# Autodesk Inventor assembly: shoot
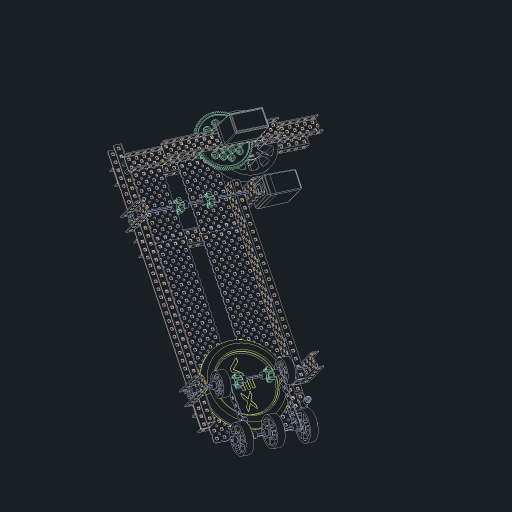
[picture p0: Inventor's stored thumbnail of the model, 512x512]
Saved by Autodesk Inventor 2023 (Build 270158000, 158)
## iProperties
Created: 2023-03-08
Part Number: shoot
Document SubType Name: Assembly
Designer: Windows Macbook
Author: Windows Macbook
## Documents named in this file (39)
- C:\Users\Windows Macbook\Desktop\VRC-SPIN-UP\Inventor\Assembly\Pre Worlds\V1\shoot.iam
- C:\Users\Windows Macbook\Desktop\VRC-SPIN-UP\Inventor\Structure\C Channel\Aluminum 1x2x1\Alu C 1x2x1x35.ipt
- C:\Users\Windows Macbook\Desktop\VRC-SPIN-UP\Inventor\Structure\C Channel\Aluminum 1x2x1\Alu C 1x2x1x14.ipt
- C:\Users\Windows Macbook\Desktop\VRC-SPIN-UP\Inventor\Structure\Plate\Steel\Steel Plate 5x25.ipt
- C:\Users\Windows Macbook\Desktop\VRC-SPIN-UP\Inventor\Structure\Plate\Steel\Steel Plate 5x10.ipt
- C:\Users\Windows Macbook\Desktop\VRC-SPIN-UP\Inventor\Structure\C Channel\Aluminum 1x2x1\Alu C 1x2x1x25.ipt
- C:\Users\Windows Macbook\Desktop\VRC-SPIN-UP\Inventor\Motion\Wheels\Flex Wheels\4 Flex, LS.iam
- C:\Users\Windows Macbook\Desktop\VRC-SPIN-UP\Inventor\Structure\Standoff\Standoff .50.ipt
- C:\Users\Windows Macbook\Desktop\VRC-SPIN-UP\Inventor\Structure\Standoff.ipt
- C:\Users\Windows Macbook\Desktop\VRC-SPIN-UP\Inventor\Structure\C Channel\Aluminum 1x3x1\Alu C 1x3x1x14.ipt
- C:\Users\Windows Macbook\Desktop\VRC-SPIN-UP\Inventor\Motion\Spacers\Spacer Nylon .375 OD\NSpacer .375 OD x .500.ipt
- C:\Users\Windows Macbook\Desktop\VRC-SPIN-UP\Inventor\Motion\Spacers\Spacer Nylon .375 OD.ipt
- C:\Users\Windows Macbook\Desktop\VRC-SPIN-UP\Inventor\Motion\Spacers\Spacer Nylon .375 OD\NSpacer .375 OD x .250.ipt
- C:\Users\Windows Macbook\Desktop\VRC-SPIN-UP\Inventor\Structure\Hardware\Screw Steel - Star.ipt
- C:\Users\Windows Macbook\Desktop\VRC-SPIN-UP\Inventor\Structure\Hardware\Screw Steel - Star\SScrew Star Smooth 1.000.ipt
- C:\Users\Windows Macbook\Desktop\VRC-SPIN-UP\Inventor\Structure\Hardware\Nut Nylock.ipt
- C:\Users\Windows Macbook\Desktop\VRC-SPIN-UP\Inventor\Motion\Shaft LS\Bearing Flat.ipt
- C:\Users\Windows Macbook\Desktop\VRC-SPIN-UP\Inventor\Motion\Spacers\Spacer Nylon .313 OD.ipt
- C:\Users\Windows Macbook\Desktop\VRC-SPIN-UP\Inventor\Motion\Gears\HS Gear\HS 12T Gear, Square.iam
- C:\Users\Windows Macbook\Desktop\VRC-SPIN-UP\Inventor\Motion\Gears\HS Gear.iam
- C:\Users\Windows Macbook\Desktop\VRC-SPIN-UP\Inventor\Motion\Gears\LS 84T Gear.ipt
- C:\Users\Windows Macbook\Desktop\VRC-SPIN-UP\Inventor\Motion\Spacers\Spacer Nylon .313 OD\NSpacer .313 OD x .125.ipt
- C:\Users\Windows Macbook\Desktop\VRC-SPIN-UP\Inventor\Motion\Spacers\Spacer Nylon .313 OD\NSpacer .313 OD x .250.ipt
- C:\Users\Windows Macbook\Desktop\VRC-SPIN-UP\Inventor\Structure\Standoff\Standoff 1.00.ipt
- C:\Users\Windows Macbook\Desktop\VRC-SPIN-UP\Inventor\Structure\C Channel\Aluminum 1x2x1\Alu C 1x2x1x15.ipt
- C:\Users\Windows Macbook\Desktop\VRC-SPIN-UP\Inventor\Structure\Plate\Steel\Steel Plate 1x8.ipt
- C:\Users\Windows Macbook\Desktop\VRC-SPIN-UP\Inventor\Disk.ipt
- C:\Users\Windows Macbook\Desktop\VRC-SPIN-UP\Inventor\Structure\C Channel\Aluminum 1x2x1\Alu C 1x2x1x5.ipt
- C:\Users\Windows Macbook\Desktop\VRC-SPIN-UP\Inventor\Motion\Shaft LS\Shaft LS\Shaft LS 8.0.ipt
- C:\Users\Windows Macbook\Desktop\VRC-SPIN-UP\Inventor\Motion\Shaft LS\Shaft LS.ipt
- C:\Users\Windows Macbook\Desktop\VRC-SPIN-UP\Inventor\Motion\Wheels\Flex Wheels\1.625 Flex, LS.iam
- C:\Users\Windows Macbook\Desktop\VRC-SPIN-UP\Inventor\Motion\Reference Files\Shaft Collar Metal.ipt
- C:\Users\Windows Macbook\Desktop\VRC-SPIN-UP\Inventor\Motion\Wheels\Flex Wheels\2 Flex, LS.iam
- C:\Users\Windows Macbook\Desktop\VRC-SPIN-UP\Inventor\Motion\Shaft LS\Shaft LS\Shaft LS 5.5.ipt
- C:\Users\Windows Macbook\Desktop\VRC-SPIN-UP\Inventor\Motion\Sprockets\9P Sprocket.iam
- C:\Users\Windows Macbook\Desktop\VRC-SPIN-UP\Inventor\Motion\Spacers\Spacer Nylon .313 OD\NSpacer .313 OD x .375.ipt
- C:\Users\Windows Macbook\Desktop\VRC-SPIN-UP\Inventor\Motion\Sprockets\9P Sprocket\9P 6T Sprocket, Square.iam
- C:\Users\Windows Macbook\Desktop\VRC-SPIN-UP\Inventor\Electronics\V5 Simple Motor.ipt
- C:\Users\Windows Macbook\Desktop\VRC-SPIN-UP\Inventor\Structure\Standoff\Standoff .75.ipt
## Components (94 placed, 31 different names)
1. Alu C 1x2x1x35:1 — Insert:1, Insert:2, Insert:15, Insert:16, Insert:18, Insert:19, Insert:22, Insert:23, Insert:43, Insert:44, Insert:91, Insert:92
2. Alu C 1x2x1x25:1 — Insert:17, Insert:113, Insert:117, Insert:118
3. Alu C 1x2x1x14:2 — Insert:1, Insert:2, Insert:7, Insert:8, Insert:9, Insert:10, Insert:24, Insert:26
4. Alu C 1x2x1x25:3 — Insert:5, Insert:6, Insert:69, Insert:70, Angle:1, Insert:96, Insert:97
5. Steel Plate 5x25:1 — Insert:9, Insert:10, Mate:1
6. Steel Plate 5x25:2 — Insert:7, Insert:8
7. Steel Plate 5x10:1
8. Steel Plate 5x10:2
9. Alu C 1x2x1x14:3 — Insert:15, Insert:16
10. 4 Flex, LS:1 [sub-assembly] — Insert:17, Insert:114
11. Standoff .75:1 — Insert:19, Insert:21
12. Standoff .75:2 — Insert:18, Insert:20
13. Alu C 1x2x1x25:2 — Insert:20, Insert:21, Insert:28, Insert:29, Insert:32, Insert:33, Insert:37, Insert:38, Insert:39, Insert:40, Insert:112
14. Alu C 1x3x1x14:1 — Insert:22, Insert:23, Insert:5, Insert:6
15. NSpacer .375 OD x .500:1 — Insert:24, Insert:25
16. NSpacer .375 OD x .250:2 — Insert:25, Insert:27
17. SScrew Star Smooth 1.000:1 — Insert:26
18. Nut Nylock:1 — Insert:27
19. Bearing Flat:1 — Insert:28, Insert:29, Insert:30
20. NSpacer .313 OD x .250:1 — Insert:30, Insert:31
21. HS 12T Gear, Square:1 [sub-assembly] — Insert:31
22. LS 84T Gear:1 — Insert:34, Insert:36
23. Bearing Flat:2 — Insert:32, Insert:33, Insert:35
24. NSpacer .313 OD x .125:2 — Insert:34, Insert:35
25. NSpacer .313 OD x .125:3 — Insert:36
26. Standoff 1.00:3 — Insert:38, Insert:41
27. Standoff 1.00:4 — Insert:37, Insert:42
28. Standoff 1.00:5 — Insert:40
29. Standoff 1.00:6 — Insert:39
30. Alu C 1x2x1x15:1 — Insert:41, Insert:42, Insert:107, Insert:108, Insert:109, Insert:111
31. Steel Plate 1x8:1 — Insert:52, Insert:53, Insert:54, Insert:56, Insert:78
32. Alu C 1x2x1x5:2 — Insert:45, Insert:46, Insert:47, Insert:48, Insert:49
33. Standoff .50:7 — Insert:44, Insert:46
34. Standoff .50:8 — Insert:43, Insert:45
35. Disk:2 — Mate:1
36. Bearing Flat:3 — Insert:47, Insert:48, Flush:1, Cylindrical:1, Insert:104
37. Shaft LS 8.0:1 — Flush:1, Cylindrical:1
38. 1.625 Flex, LS:1 [sub-assembly] — Insert:49, Insert:50, Insert:56
39. Shaft Collar Metal:1 — Insert:50
40. 2 Flex, LS:1 [sub-assembly] — Insert:52, Insert:58
41. Shaft Collar Metal:2 — Insert:55, Insert:76
42. Bearing Flat:4 — Insert:53, Insert:54, Insert:55
43. NSpacer .313 OD x .375:5 — Insert:78, Insert:79
44. Shaft Collar Metal:4 — Insert:58, Flush:2, Cylindrical:2
45. Steel Plate 1x8:2 — Insert:77
46. 1.625 Flex, LS:2 [sub-assembly] — Insert:72, Insert:73
47. 2 Flex, LS:2 [sub-assembly] — Insert:66
48. Shaft Collar Metal:6
49. Bearing Flat:5
50. NSpacer .313 OD x .375:4 — Insert:77, Insert:80
51. Shaft Collar Metal:8 — Insert:66, Cylindrical:3
52. Alu C 1x2x1x5:3 — Insert:71, Angle:1, Insert:72
53. Bearing Flat:6 — Insert:103
54. Standoff .50:9 — Insert:69
55. Standoff .50:10 — Insert:70, Insert:71
56. Shaft Collar Metal:9 — Insert:73
57. Shaft LS 5.5:2 — Flush:2, Cylindrical:2, Cylindrical:3
58. 2 Flex, LS:3 [sub-assembly] — Insert:74, Insert:75
59. Shaft Collar Metal:10 — Insert:75
60. Shaft Collar Metal:11 — Insert:74, Insert:76
61. 9P 6T Sprocket, Square:1 [sub-assembly] — Insert:79, Insert:82
62. 9P 6T Sprocket, Square:2 [sub-assembly] — Insert:80, Insert:81
63. Shaft Collar Metal:12 — Insert:82
64. Shaft Collar Metal:13 — Insert:81
65. Alu C 1x2x1x5:4 — Insert:95
66. Standoff .50:11 — Insert:92
67. Standoff .50:12 — Insert:91
68. Bearing Flat:7 — Insert:101
69. Shaft LS 8.0:3
70. Alu C 1x2x1x5:5 — Insert:90, Insert:100
71. Bearing Flat:8 — Insert:105, Insert:106, Insert:110
72. Standoff .50:13 — Insert:90, Insert:97
73. Standoff .50:14 — Insert:96
74. 9P 6T Sprocket, Square:3 [sub-assembly] — Insert:94
75. Shaft Collar Metal:14
76. Shaft Collar Metal:15 — Insert:94, Insert:95
77. 9P 6T Sprocket, Square:4 [sub-assembly]
78. Shaft Collar Metal:16 — Insert:100
79. Shaft Collar Metal:17
80. Shaft Collar Metal:19 — Insert:103
81. Shaft Collar Metal:20 — Insert:101
82. Shaft Collar Metal:21 — Insert:104
83. V5 Simple Motor:1 — Insert:105, Insert:106
84. V5 Simple Motor:2 — Insert:107, Insert:108
85. Shaft Collar Metal:22 — Insert:109
86. Shaft Collar Metal:23 — Insert:110
87. Shaft Collar Metal:24 — Insert:113
88. Shaft Collar Metal:25 — Insert:112
89. Shaft Collar Metal:26 — Insert:111
90. NSpacer .313 OD x .250:6 — Insert:114
91. Standoff 1.00:15 — Insert:115
92. Standoff .75:16 — Insert:115, Insert:118
93. Standoff 1.00:17
94. Standoff .75:18 — Insert:117
## Relationships (122: Insert 113, CylindricalJoint 4, Flush 3, Mate 1, Angle 1)
- Insert:1: Alu C 1x2x1x35:1 ↔ Alu C 1x2x1x14:2
- Insert:2: Alu C 1x2x1x35:1 ↔ Alu C 1x2x1x14:2
- [Insert]: Alu C 1x2x1x35:1 ↔ Alu C 1x2x1x25:1
- [Insert]: Alu C 1x2x1x35:1 ↔ Alu C 1x2x1x25:1
- Insert:5: Alu C 1x2x1x25:3 ↔ Alu C 1x3x1x14:1
- Insert:6: Alu C 1x2x1x25:3 ↔ Alu C 1x3x1x14:1
- Insert:7: Alu C 1x2x1x14:2 ↔ Steel Plate 5x25:2
- Insert:8: Alu C 1x2x1x14:2 ↔ Steel Plate 5x25:2
- Insert:9: Alu C 1x2x1x14:2 ↔ Steel Plate 5x25:1
- Insert:10: Alu C 1x2x1x14:2 ↔ Steel Plate 5x25:1
- [Insert]: Alu C 1x2x1x25:1 ↔ Steel Plate 5x10:1
- [Insert]: Alu C 1x2x1x25:1 ↔ Steel Plate 5x10:1
- [Insert]: Alu C 1x2x1x25:1 ↔ Steel Plate 5x10:2
- [Insert]: Alu C 1x2x1x25:1 ↔ Steel Plate 5x10:2
- Insert:15: Alu C 1x2x1x35:1 ↔ Alu C 1x2x1x14:3
- Insert:16: Alu C 1x2x1x35:1 ↔ Alu C 1x2x1x14:3
- Insert:17: Alu C 1x2x1x25:1 ↔ 4 Flex, LS:1
- Insert:18: Alu C 1x2x1x35:1 ↔ Standoff .75:2
- Insert:19: Alu C 1x2x1x35:1 ↔ Standoff .75:1
- Insert:20: Standoff .75:2 ↔ Alu C 1x2x1x25:2
- Insert:21: Standoff .75:1 ↔ Alu C 1x2x1x25:2
- Insert:22: Alu C 1x2x1x35:1 ↔ Alu C 1x3x1x14:1
- Insert:23: Alu C 1x2x1x35:1 ↔ Alu C 1x3x1x14:1
- Insert:24: Alu C 1x2x1x14:2 ↔ NSpacer .375 OD x .500:1
- Insert:25: NSpacer .375 OD x .500:1 ↔ NSpacer .375 OD x .250:2
- Insert:26: Alu C 1x2x1x14:2 ↔ SScrew Star Smooth 1.000:1
- Insert:27: NSpacer .375 OD x .250:2 ↔ Nut Nylock:1
- Insert:28: Alu C 1x2x1x25:2 ↔ Bearing Flat:1
- Insert:29: Alu C 1x2x1x25:2 ↔ Bearing Flat:1
- Insert:30: Bearing Flat:1 ↔ NSpacer .313 OD x .250:1
- Insert:31: NSpacer .313 OD x .250:1 ↔ HS 12T Gear, Square:1
- Insert:32: Alu C 1x2x1x25:2 ↔ Bearing Flat:2
- Insert:33: Alu C 1x2x1x25:2 ↔ Bearing Flat:2
- Insert:34: LS 84T Gear:1 ↔ NSpacer .313 OD x .125:2
- Insert:35: Bearing Flat:2 ↔ NSpacer .313 OD x .125:2
- Insert:36: LS 84T Gear:1 ↔ NSpacer .313 OD x .125:3
- Insert:37: Alu C 1x2x1x25:2 ↔ Standoff 1.00:4
- Insert:38: Alu C 1x2x1x25:2 ↔ Standoff 1.00:3
- Insert:39: Alu C 1x2x1x25:2 ↔ Standoff 1.00:6
- Insert:40: Alu C 1x2x1x25:2 ↔ Standoff 1.00:5
- Insert:41: Standoff 1.00:3 ↔ Alu C 1x2x1x15:1
- Insert:42: Standoff 1.00:4 ↔ Alu C 1x2x1x15:1
- Insert:43: Alu C 1x2x1x35:1 ↔ Standoff .50:8
- Insert:44: Alu C 1x2x1x35:1 ↔ Standoff .50:7
- Insert:45: Alu C 1x2x1x5:2 ↔ Standoff .50:8
- Insert:46: Alu C 1x2x1x5:2 ↔ Standoff .50:7
- Mate:1: Steel Plate 5x25:1 ↔ Disk:2
- Insert:47: Alu C 1x2x1x5:2 ↔ Bearing Flat:3
- Insert:48: Alu C 1x2x1x5:2 ↔ Bearing Flat:3
- Flush:1: Bearing Flat:3 ↔ Shaft LS 8.0:1
- Cylindrical:1: Bearing Flat:3 ↔ Shaft LS 8.0:1
- Insert:49 (25.4 mm): Alu C 1x2x1x5:2 ↔ 1.625 Flex, LS:1
- Insert:50: 1.625 Flex, LS:1 ↔ Shaft Collar Metal:1
- Insert:52: Steel Plate 1x8:1 ↔ 2 Flex, LS:1
- Insert:53: Steel Plate 1x8:1 ↔ Bearing Flat:4
- Insert:54: Steel Plate 1x8:1 ↔ Bearing Flat:4
- Insert:55: Shaft Collar Metal:2 ↔ Bearing Flat:4
- Insert:56: Steel Plate 1x8:1 ↔ 1.625 Flex, LS:1
- Insert:58: 2 Flex, LS:1 ↔ Shaft Collar Metal:4
- [Insert]: Steel Plate 1x8:2 ↔ 2 Flex, LS:2
- [Insert]: Steel Plate 1x8:2 ↔ Bearing Flat:5
- [Insert]: Steel Plate 1x8:2 ↔ Bearing Flat:5
- [Insert]: Shaft Collar Metal:6 ↔ Bearing Flat:5
- [Insert]: Steel Plate 1x8:2 ↔ 1.625 Flex, LS:2
- Insert:66: 2 Flex, LS:2 ↔ Shaft Collar Metal:8
- [Insert]: Alu C 1x2x1x5:3 ↔ Bearing Flat:6
- [Insert]: Alu C 1x2x1x5:3 ↔ Bearing Flat:6
- Insert:69: Alu C 1x2x1x25:3 ↔ Standoff .50:9
- Insert:70: Alu C 1x2x1x25:3 ↔ Standoff .50:10
- Insert:71: Alu C 1x2x1x5:3 ↔ Standoff .50:10
- Angle:1 (0 deg): Alu C 1x2x1x25:3 ↔ Alu C 1x2x1x5:3
- Insert:72 (25.4 mm): 1.625 Flex, LS:2 ↔ Alu C 1x2x1x5:3
- Insert:73: 1.625 Flex, LS:2 ↔ Shaft Collar Metal:9
- Flush:2: Shaft Collar Metal:4 ↔ Shaft LS 5.5:2
- Cylindrical:2: Shaft Collar Metal:4 ↔ Shaft LS 5.5:2
- Cylindrical:3: Shaft Collar Metal:8 ↔ Shaft LS 5.5:2
- Insert:74: 2 Flex, LS:3 ↔ Shaft Collar Metal:11
- Insert:75: 2 Flex, LS:3 ↔ Shaft Collar Metal:10
- Insert:76 (12.7 mm): Shaft Collar Metal:2 ↔ Shaft Collar Metal:11
- Insert:77: Steel Plate 1x8:2 ↔ NSpacer .313 OD x .375:4
- Insert:78: Steel Plate 1x8:1 ↔ NSpacer .313 OD x .375:5
- Insert:79: NSpacer .313 OD x .375:5 ↔ 9P 6T Sprocket, Square:1
- Insert:80: NSpacer .313 OD x .375:4 ↔ 9P 6T Sprocket, Square:2
- Insert:81: 9P 6T Sprocket, Square:2 ↔ Shaft Collar Metal:13
- Insert:82: 9P 6T Sprocket, Square:1 ↔ Shaft Collar Metal:12
- [Insert]: Alu C 1x2x1x5:4 ↔ Standoff .50:12
- [Insert]: Alu C 1x2x1x5:4 ↔ Standoff .50:11
- [Insert]: Alu C 1x2x1x5:4 ↔ Bearing Flat:7
- [Insert]: Alu C 1x2x1x5:4 ↔ Bearing Flat:7
- [Flush]: Bearing Flat:7 ↔ Shaft LS 8.0:3
- [CylindricalJoint]: Bearing Flat:7 ↔ Shaft LS 8.0:3
- [Insert]: Alu C 1x2x1x5:5 ↔ Bearing Flat:8
- [Insert]: Alu C 1x2x1x5:5 ↔ Bearing Flat:8
- [Insert]: Alu C 1x2x1x5:5 ↔ Standoff .50:14
- Insert:90: Alu C 1x2x1x5:5 ↔ Standoff .50:13
- Insert:91: Alu C 1x2x1x35:1 ↔ Standoff .50:12
- Insert:92: Alu C 1x2x1x35:1 ↔ Standoff .50:11
- [Insert]: 9P 6T Sprocket, Square:3 ↔ Shaft Collar Metal:14
- Insert:94: 9P 6T Sprocket, Square:3 ↔ Shaft Collar Metal:15
- Insert:95 (50.8 mm): Alu C 1x2x1x5:4 ↔ Shaft Collar Metal:15
- Insert:96: Alu C 1x2x1x25:3 ↔ Standoff .50:14
- Insert:97: Alu C 1x2x1x25:3 ↔ Standoff .50:13
- [Insert]: 9P 6T Sprocket, Square:4 ↔ Shaft Collar Metal:16
- [Insert]: 9P 6T Sprocket, Square:4 ↔ Shaft Collar Metal:17
- Insert:100 (50.8 mm): Alu C 1x2x1x5:5 ↔ Shaft Collar Metal:16
- Insert:101: Bearing Flat:7 ↔ Shaft Collar Metal:20
- Insert:103: Bearing Flat:6 ↔ Shaft Collar Metal:19
- Insert:104: Bearing Flat:3 ↔ Shaft Collar Metal:21
- Insert:105: Bearing Flat:8 ↔ V5 Simple Motor:1
- Insert:106: Bearing Flat:8 ↔ V5 Simple Motor:1
- Insert:107: Alu C 1x2x1x15:1 ↔ V5 Simple Motor:2
- Insert:108: Alu C 1x2x1x15:1 ↔ V5 Simple Motor:2
- Insert:109: Alu C 1x2x1x15:1 ↔ Shaft Collar Metal:22
- Insert:110: Bearing Flat:8 ↔ Shaft Collar Metal:23
- Insert:111: Alu C 1x2x1x15:1 ↔ Shaft Collar Metal:26
- Insert:112: Alu C 1x2x1x25:2 ↔ Shaft Collar Metal:25
- Insert:113: Alu C 1x2x1x25:1 ↔ Shaft Collar Metal:24
- Insert:114: 4 Flex, LS:1 ↔ NSpacer .313 OD x .250:6
- Insert:115: Standoff 1.00:15 ↔ Standoff .75:16
- [Insert]: Standoff 1.00:17 ↔ Standoff .75:18
- Insert:117: Alu C 1x2x1x25:1 ↔ Standoff .75:18
- Insert:118: Alu C 1x2x1x25:1 ↔ Standoff .75:16
## Named parameters: d65_d57 = 0 mm, d66_d58 = 0 mm, d67_d59 = 0 mm, d68_d60 = 0 mm, d69_d61 = 0 mm, d72_d49 = 0 mm, d73_d50 = 0 mm, d95_d46 = 0 mm, d96_d47 = 0 mm, d97_d49 = 0 mm, d98_d50 = 0 mm, d99_d51 = 0 mm, d100_d52 = 141.83556 deg, d101_d77 = 0 mm, d102_d53 = 0 mm, d103_d72_d49 = 0 mm, d104_d73_d50 = 0 mm, d108_d94 = 0 mm, d113_d108_d94 = 0 mm, d114_d109 = 0 mm, d131_d130 = 0 mm
